# Autodesk Inventor assembly: Assembly_Cube_Lens_Cylindrical__cheap_v3
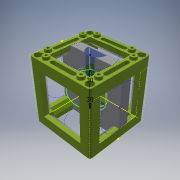
[picture p0: Inventor's stored thumbnail of the model, 180x180]
Saved by Autodesk Inventor 2019 (Build 230136000, 136)
## iProperties
Created: 2021-02-17
Part Number: Assembly_Cube_Lens_Cylindrical__cheap_v3
Document SubType Name: Assembly
Designer: marsikovabarbora
Author: marsikovabarbora
## Documents named in this file (4)
- C:\Users\marsikovabarbora\Dropbox\UC2\02_CAD\INVENTOR\uc2_v3\Assembly_Cube_Lens_Cylindrical__cheap_v3.iam
- C:\Users\marsikovabarbora\Dropbox\UC2\02_CAD\INVENTOR\uc2_v3\Assembly_Cube_empty_IM_v3.iam
- C:\Users\marsikovabarbora\Dropbox\UC2\02_CAD\INVENTOR\uc2_v3\00_Glassslab_Lens_Cylindrical_30mm_Plexiglas.ipt
- C:\Users\marsikovabarbora\Dropbox\UC2\02_CAD\INVENTOR\uc2_v3\20_Cube_Insert_Lens_Cylindrical_Plexiglas_glassslab_v3.ipt
## Components (3 placed, 3 different names)
1. Assembly_Cube_empty_IM_v3:1 [sub-assembly] — Flush:1, Flush:2, Mate:1, Flush:3, Flush:4, Mate:5
2. 00_Glassslab_Lens_Cylindrical_30mm_Plexiglas:1 — Mate:2, Mate:3, Mate:4
3. 20_Cube_Insert_Lens_Cylindrical_Plexiglas_glassslab_v3:1 — Mate:2, Mate:3, Mate:4, Flush:3, Flush:4, Mate:5
## Relationships (9: Mate 5, Flush 4)
- Flush:1: Assembly_Cube_empty_IM_v3:1
- Flush:2: Assembly_Cube_empty_IM_v3:1
- Mate:1: Assembly_Cube_empty_IM_v3:1
- Mate:2: 00_Glassslab_Lens_Cylindrical_30mm_Plexiglas:1 ↔ 20_Cube_Insert_Lens_Cylindrical_Plexiglas_glassslab_v3:1
- Mate:3: 00_Glassslab_Lens_Cylindrical_30mm_Plexiglas:1 ↔ 20_Cube_Insert_Lens_Cylindrical_Plexiglas_glassslab_v3:1
- Mate:4: 00_Glassslab_Lens_Cylindrical_30mm_Plexiglas:1 ↔ 20_Cube_Insert_Lens_Cylindrical_Plexiglas_glassslab_v3:1
- Flush:3: Assembly_Cube_empty_IM_v3:1 ↔ 20_Cube_Insert_Lens_Cylindrical_Plexiglas_glassslab_v3:1
- Flush:4: Assembly_Cube_empty_IM_v3:1 ↔ 20_Cube_Insert_Lens_Cylindrical_Plexiglas_glassslab_v3:1
- Mate:5: Assembly_Cube_empty_IM_v3:1 ↔ 20_Cube_Insert_Lens_Cylindrical_Plexiglas_glassslab_v3:1
